# Autodesk Inventor assembly: Beam Break & Magnetic Limit Switch Universal Mount
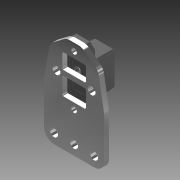
[picture p0: Inventor's stored thumbnail of the model, 180x180]
Saved by Autodesk Inventor 2022 (Build 260153000, 153)
## iProperties
Created: 2022-02-13
Part Number: Beam Break & Magnetic Limit Switch Universal Mount
Document SubType Name: Assembly
Designer: Desktop
Author: Desktop
## iProperties of the stored document MemberDocs/x4xecfuxhPswgrof51oflgtr3Wc
Created: 2022-02-13
Part Number: Beam Break & Magnetic Limit Switch Universal Mount
Document SubType Name: Assembly
Designer: Desktop
Author: Desktop
## iProperties of the stored document MemberDocs/x2spaeqedEsmptqemDhmvbjxw0f
Created: 2022-02-13
Part Number: Beam Break & Magnetic Limit Switch Universal Mount
Document SubType Name: Assembly
Designer: Desktop
Author: Desktop
## iProperties of the stored document MemberDocs/xWznkrp5uOsul3uxoIob5mzqcMa
Created: 2022-02-13
Part Number: Beam Break & Magnetic Limit Switch Universal Mount
Document SubType Name: Assembly
Designer: Desktop
Author: Desktop
## iProperties of the stored document MemberDocs/xMclvntcpA0q2tg40CiklaxmaLe
Created: 2022-02-13
Part Number: Beam Break & Magnetic Limit Switch Universal Mount
Document SubType Name: Assembly
Designer: Desktop
Author: Desktop
## Documents named in this file (13)
- E:\Middleton Robotics\Collaborative Robots\Collaborative Part Library\Electronics\FRC\Sensors\Beam Break & Magnetic Limit Switch Universal Mount.iam
- E:\Middleton Robotics\Collaborative Robots\Collaborative Part Library\Standard Custom Parts\Plates\Standard Sensor Mount.ipt
- E:\Middleton Robotics\Collaborative Robots\Collaborative Part Library\Electronics\FRC\Sensors\Rev Magnetic Limit Switch REV-40-1465.ipt
- E:\Middleton Robotics\Collaborative Robots\Collaborative Part Library\Electronics\FRC\Sensors\Adafruit Beam Break Cover.ipt
- E:\Middleton Robotics\Collaborative Robots\Collaborative Part Library\Electronics\FRC\Sensors\IR Break Beam Sensor - 5mm LEDs v3.ipt
- E:\Middleton Robotics\Collaborative Robots\Collaborative Part Library\Hardware\Fasteners\Machine Screws.ipt
- E:\Middleton Robotics\Collaborative Robots\Collaborative Part Library\Hardware\Nuts and Threaded Blocks\Nuts.ipt
- E:\Middleton Robotics\Collaborative Robots\Collaborative Part Library\Hardware\Fasteners\Rivet.ipt
- E:\Middleton Robotics\Collaborative Robots\Collaborative Part Library\Hardware\Nuts and Threaded Blocks\Nuts\6-32 Pan Head Nylon locknut.ipt
- E:\Middleton Robotics\Collaborative Robots\Collaborative Part Library\Hardware\Fasteners\Machine Screws\6-32 UNCx0.375 Socket Head Cap Screw.ipt
- E:\Middleton Robotics\Collaborative Robots\Collaborative Part Library\Hardware\Nuts and Threaded Blocks\Nuts\10-32 Pan Head Nylon locknut.ipt
- E:\Middleton Robotics\Collaborative Robots\Collaborative Part Library\Hardware\Fasteners\Machine Screws\10-32 UNFx0.5 Socket Head Cap Screw.ipt
- E:\Middleton Robotics\Collaborative Robots\Collaborative Part Library\Hardware\Fasteners\Machine Screws\6-32 UNCx0.5 Socket Head Cap Screw.ipt
## Components (4 placed, 4 different names)
1. Standard Sensor Mount:1 — Insert:1, Mate:4, Insert:2, Insert:3, Flush:1, Flush:2, Flush:3
2. Rev Magnetic Limit Switch REV-40-1465:1 — Insert:2, Insert:3
3. Adafruit Beam Break Cover:1 — Insert:1, Mate:4
4. IR Break Beam Sensor - 5mm LEDs v3:1
## Relationships (10: Mate 4, Insert 3, Flush 3)
- [Mate]: Adafruit Beam Break Cover:1 ↔ IR Break Beam Sensor - 5mm LEDs v3:1
- [Mate]: Adafruit Beam Break Cover:1 ↔ IR Break Beam Sensor - 5mm LEDs v3:1
- [Mate]: Adafruit Beam Break Cover:1 ↔ IR Break Beam Sensor - 5mm LEDs v3:1
- Insert:1: Standard Sensor Mount:1 ↔ Adafruit Beam Break Cover:1
- Mate:4: Standard Sensor Mount:1 ↔ Adafruit Beam Break Cover:1
- Insert:2: Standard Sensor Mount:1 ↔ Rev Magnetic Limit Switch REV-40-1465:1
- Insert:3: Standard Sensor Mount:1 ↔ Rev Magnetic Limit Switch REV-40-1465:1
- Flush:1: Standard Sensor Mount:1
- Flush:2: Standard Sensor Mount:1
- Flush:3: Standard Sensor Mount:1
